# Autodesk Inventor assembly: Ensamblaje1
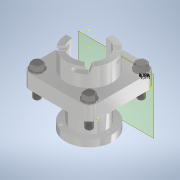
[picture p0: Inventor's stored thumbnail of the model, 180x180]
Saved by Autodesk Inventor 2020.2 (Build 242310000, 310)
## iProperties
Created: 2020-04-23
Part Number: Ensamblaje1
Document SubType Name: Assembly
Designer: Luis Carlos Gallardo
Author: Luis Carlos Gallardo
## Documents named in this file (4)
- C:\Users\Luis Carlos Gallardo\Desktop\Examen Unidad I INVENTOR\23.XX\Ensamblaje1.iam
- C:\Users\Luis Carlos Gallardo\Desktop\Examen Unidad I INVENTOR\23.XX\pieza 23.xx.1.ipt
- C:\Users\Luis Carlos Gallardo\Desktop\Examen Unidad I INVENTOR\23.XX\pieza 23.xx.2.ipt
- C:\Users\Luis Carlos Gallardo\Documents\Inventor\Content Center Files\R2020\es-ES\AS 1427(00)\AS 1427 - M8 x 30(4).ipt
## Components (5 placed, 3 different names)
1. pieza 23.xx.1:1 — Coincidencia:1, Coincidencia:2, Coincidencia:3, Coincidencia:4, Coincidencia:5, Coincidencia:6, Coincidencia:7
2. pieza 23.xx.2:1 — Coincidencia:1
3. AS 1427 - Métrico M8 x 30:1 — Coincidencia:2, Coincidencia:3
4. AS 1427 - Métrico M8 x 30:2 — Coincidencia:4, Coincidencia:5
5. AS 1427 - Métrico M8 x 30:3 — Coincidencia:6, Coincidencia:7
## Relationships (7: Mate 7)
- Coincidencia:1 [Mate]: pieza 23.xx.1:1 ↔ pieza 23.xx.2:1
- Coincidencia:2 [Mate]: pieza 23.xx.1:1 ↔ AS 1427 - Métrico M8 x 30:1
- Coincidencia:3 [Mate]: pieza 23.xx.1:1 ↔ AS 1427 - Métrico M8 x 30:1
- Coincidencia:4 [Mate]: pieza 23.xx.1:1 ↔ AS 1427 - Métrico M8 x 30:2
- Coincidencia:5 [Mate]: pieza 23.xx.1:1 ↔ AS 1427 - Métrico M8 x 30:2
- Coincidencia:6 [Mate]: pieza 23.xx.1:1 ↔ AS 1427 - Métrico M8 x 30:3
- Coincidencia:7 [Mate]: pieza 23.xx.1:1 ↔ AS 1427 - Métrico M8 x 30:3
